# Autodesk Inventor assembly: ArianSat-Stratosphere
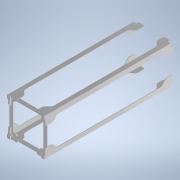
[picture p0: Inventor's stored thumbnail of the model, 180x180]
Saved by Autodesk Inventor 2022 (Build 260153000, 153)
## iProperties
Created: 2021-11-12
Part Number: ArianSat-Stratosphere
Document SubType Name: Assembly
Designer: Sergey
Author: Sergey
## Documents named in this file (3)
- C:\!MEGA\!myFiles\ArianSat-Stratosphere\Structural\ArianSat-Stratosphere.iam
- C:\!MEGA\!myFiles\ArianSat-Stratosphere\Structural\Parts\Other\aluminium corner 25x25x1,2.ipt
- C:\!MEGA\!myFiles\ArianSat-Stratosphere\Structural\Parts\Other\BottomPlate.ipt
## Components (5 placed, 2 different names)
1. aluminium corner 25x25x1,2:1 — Rotational:1, Mate:3
2. aluminium corner 25x25x1,2:2 — Rotational:3, Mate:6
3. aluminium corner 25x25x1,2:3 — Rotational:4, Mate:4, Mate:7
4. aluminium corner 25x25x1,2:4 — Rotational:2, Mate:5, Mate:8
5. BottomPlate:1 — Rotational:1, Rotational:2, Rotational:3, Rotational:4, Mate:3, Mate:4, Mate:5, Mate:6, Mate:9
## Relationships (11: Mate 7, RevoluteJoint 4)
- Rotational:1 [RevoluteJoint]: aluminium corner 25x25x1,2:1 ↔ BottomPlate:1
- Rotational:2 [RevoluteJoint]: aluminium corner 25x25x1,2:4 ↔ BottomPlate:1
- Rotational:3 [RevoluteJoint]: aluminium corner 25x25x1,2:2 ↔ BottomPlate:1
- Rotational:4 [RevoluteJoint]: aluminium corner 25x25x1,2:3 ↔ BottomPlate:1
- Mate:3: aluminium corner 25x25x1,2:1 ↔ BottomPlate:1
- Mate:4: aluminium corner 25x25x1,2:3 ↔ BottomPlate:1
- Mate:5: aluminium corner 25x25x1,2:4 ↔ BottomPlate:1
- Mate:6: aluminium corner 25x25x1,2:2 ↔ BottomPlate:1
- Mate:7: aluminium corner 25x25x1,2:3
- Mate:8: aluminium corner 25x25x1,2:4
- Mate:9: BottomPlate:1
